# Autodesk Inventor assembly: MotorChainV4
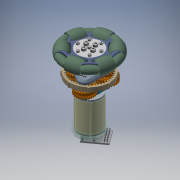
[picture p0: Inventor's stored thumbnail of the model, 180x180]
Saved by Autodesk Inventor 2019.1 (Build 231200000, 200)
## iProperties
Created: 2019-01-03
Part Number: MotorChainV4
Material: Generisch
Document SubType Name: Assembly
Designer: JochenAlt
Author: JochenAlt
## Documents named in this file (12)
- D:\Projects\Ondine\CAD\PlanetaryGear2\MotorChainV4.iam
- D:\Projects\Ondine\CAD\PlanetaryGear2\PlanetaryGearConstruction\PlanetaryGear2.iam
- D:\Projects\Ondine\CAD\Maxxon Motor 272766.ipt
- D:\Projects\Ondine\CAD\Encoder\MagneticEncoder V2.iam
- D:\Projects\Ondine\CAD\Bearings\AST_Bearings_SMR74.ipt
- D:\Projects\Ondine\CAD\PlanetaryGear2\OmniWheelAxisV2.ipt
- D:\Projects\Ondine\CAD\PlanetaryGear2\GearAxisSleeve.ipt
- D:\Projects\Ondine\CAD\OmniWheel.iam
- D:\Projects\Ondine\CAD\Bearings\W 637_4 X-2Z.iam
- D:\Projects\Ondine\CAD\PlanetaryGear2\OmniWheelSleeve1.ipt
- D:\Projects\Ondine\CAD\PlanetaryGear2\OmniWheelSleeve2.ipt
- C:\Users\JochenAlt\Documents\Inventor\Content Center Files\R2019\de-DE\DIN 912\DIN 912 - M2,5 x 0,45 x 8 x 6,875.ipt
## Components (14 placed, 11 different names)
1. PlanetaryGear2:1 [sub-assembly] — Passend:1, Passend:2, Passend:5, Passend:6, Passend:7, Passend:10, Passend:17, Passend:22, Drehung:1, Passend:23, Passend:24, Passend:25, Passend:26, Passend:27, Passend:28, Passend:29, Passend:30
2. Maxxon Motor 272766:1 — Passend:1, Passend:2, Passend:3, Passend:4
3. EncoderedMotorV2:1 [sub-assembly] — Passend:3, Passend:4
4. AST_Bearings_SMR74:1 — Passend:5, Passend:6, Passend:8, Passend:22
5. OmniWheelAxisSmall:1 — Passend:7, Passend:8, Passend:9, Passend:11, Passend:15, Passend:16, Passend:18
6. SunBushing:1 — Passend:9, Passend:10
7. OmniWheel:1 [sub-assembly] — Passend:11, Passend:19, Drehung:1
8. W 637_4 X-2Z:1 [sub-assembly] — Passend:15, Passend:20, Passend:21
9. OmniWheelBushing:1 — Passend:18, Passend:19, Passend:20
10. BottomBushing:1 — Passend:16, Passend:17, Passend:21
11. DIN 912 - ersetzt durch DIN EN ISO 4762 M2,5 x 8:1 — Passend:23, Passend:24
12. DIN 912 - ersetzt durch DIN EN ISO 4762 M2,5 x 8:2 — Passend:25, Passend:26
13. DIN 912 - ersetzt durch DIN EN ISO 4762 M2,5 x 8:3 — Passend:27, Passend:28
14. DIN 912 - ersetzt durch DIN EN ISO 4762 M2,5 x 8:4 — Passend:29, Passend:30
## Relationships (28: Mate 27, RelateRotation 1)
- Passend:1 [Mate]: PlanetaryGear2:1 ↔ Maxxon Motor 272766:1
- Passend:2 [Mate] (0.5 mm): PlanetaryGear2:1 ↔ Maxxon Motor 272766:1
- Passend:3 [Mate]: Maxxon Motor 272766:1 ↔ EncoderedMotorV2:1
- Passend:4 [Mate]: Maxxon Motor 272766:1 ↔ EncoderedMotorV2:1
- Passend:5 [Mate]: PlanetaryGear2:1 ↔ AST_Bearings_SMR74:1
- Passend:6 [Mate]: PlanetaryGear2:1 ↔ AST_Bearings_SMR74:1
- Passend:7 [Mate]: PlanetaryGear2:1 ↔ OmniWheelAxisSmall:1
- Passend:8 [Mate]: AST_Bearings_SMR74:1 ↔ OmniWheelAxisSmall:1
- Passend:9 [Mate]: OmniWheelAxisSmall:1 ↔ SunBushing:1
- Passend:10 [Mate]: PlanetaryGear2:1 ↔ SunBushing:1
- Passend:11 [Mate]: OmniWheelAxisSmall:1 ↔ OmniWheel:1
- Passend:15 [Mate]: OmniWheelAxisSmall:1 ↔ W 637_4 X-2Z:1
- Passend:16 [Mate]: OmniWheelAxisSmall:1 ↔ BottomBushing:1
- Passend:17 [Mate]: PlanetaryGear2:1 ↔ BottomBushing:1
- Passend:18 [Mate]: OmniWheelAxisSmall:1 ↔ OmniWheelBushing:1
- Passend:19 [Mate]: OmniWheel:1 ↔ OmniWheelBushing:1
- Passend:20 [Mate]: W 637_4 X-2Z:1 ↔ OmniWheelBushing:1
- Passend:21 [Mate]: W 637_4 X-2Z:1 ↔ BottomBushing:1
- Passend:22 [Mate]: PlanetaryGear2:1 ↔ AST_Bearings_SMR74:1
- Drehung:1 [RelateRotation] (-1 ul): PlanetaryGear2:1 ↔ OmniWheel:1
- Passend:23 [Mate]: PlanetaryGear2:1 ↔ DIN 912 - ersetzt durch DIN EN ISO 4762 M2,5 x 8:1
- Passend:24 [Mate]: PlanetaryGear2:1 ↔ DIN 912 - ersetzt durch DIN EN ISO 4762 M2,5 x 8:1
- Passend:25 [Mate]: PlanetaryGear2:1 ↔ DIN 912 - ersetzt durch DIN EN ISO 4762 M2,5 x 8:2
- Passend:26 [Mate]: PlanetaryGear2:1 ↔ DIN 912 - ersetzt durch DIN EN ISO 4762 M2,5 x 8:2
- Passend:27 [Mate]: PlanetaryGear2:1 ↔ DIN 912 - ersetzt durch DIN EN ISO 4762 M2,5 x 8:3
- Passend:28 [Mate]: PlanetaryGear2:1 ↔ DIN 912 - ersetzt durch DIN EN ISO 4762 M2,5 x 8:3
- Passend:29 [Mate]: PlanetaryGear2:1 ↔ DIN 912 - ersetzt durch DIN EN ISO 4762 M2,5 x 8:4
- Passend:30 [Mate]: PlanetaryGear2:1 ↔ DIN 912 - ersetzt durch DIN EN ISO 4762 M2,5 x 8:4
